# Autodesk Inventor assembly: Intake Pivot Encoder Mount
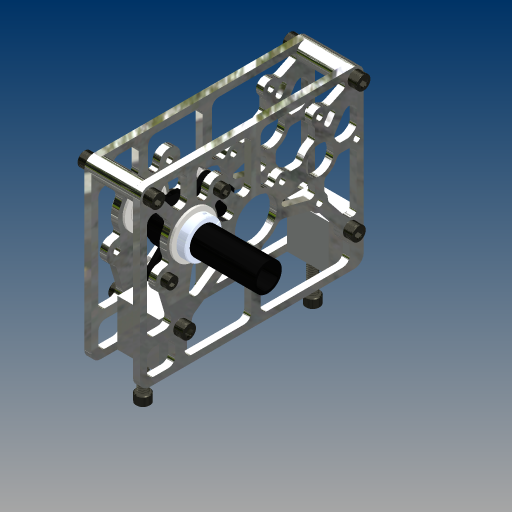
[picture p0: Inventor's stored thumbnail of the model, 512x512]
Saved by Autodesk Inventor 2024.3 (Build 283343000, 343)
## iProperties
Created: 2024-08-03
Part Number: Intake Pivot Encoder Mount
Document SubType Name: Assembly
Designer: Kenji
Author: Kenji
## Documents named in this file (15)
- C:\Users\Kenji\Documents\GitHub\1622-2024-Summer-CAD-A-Thon\Intake\Intake Pivot Encoder Mount.iam
- C:\Users\Kenji\Documents\GitHub\1622-2024-Summer-CAD-A-Thon\Intake\Intake Pivot Gearbox Plate.ipt
- C:\Users\Kenji\Documents\GitHub\1622-2024-Summer-CAD-A-Thon\Intake\Intake Pivot Spacer 3.ipt
- C:\Users\Kenji\Documents\GitHub\1622-2024-Summer-CAD-A-Thon\Intake\Intake Pivot Billet.ipt
- C:\Users\Kenji\Documents\GitHub\1622-2024-Summer-CAD-A-Thon\COTS Library\Fasteners\Bolts\Socket-Head\0.25-20\COTS_91251A539_Black-Oxide Alloy Steel Socket Head Screw (1).ipt
- C:\Users\Kenji\Documents\GitHub\1622-2024-Summer-CAD-A-Thon\COTS Library\Motion\Bearings\COTS_WCP-0783_1.125ODHexBearing.ipt
- C:\Users\Kenji\Documents\GitHub\1622-2024-Summer-CAD-A-Thon\COTS Library\Fasteners\Bolts\Button-Head\0.25-20\COTS_0.25-20_ButtonHead_0.5inlong_StainlessSteel_92949A537.ipt
- C:\Users\Kenji\Documents\GitHub\1622-2024-Summer-CAD-A-Thon\COTS Library\Fasteners\Washers\COTS_90107A029_316 Stainless Steel Washer.ipt
- C:\Users\Kenji\Documents\GitHub\1622-2024-Summer-CAD-A-Thon\Intake\REV-11-1271(ThroughBoreEncoder).iam
- C:\Users\Kenji\Documents\GitHub\1622-2024-Summer-CAD-A-Thon\COTS Library\Fasteners\Nuts\COTS_90631A411_10-32_Nylock_Nut.ipt
- C:\Users\Kenji\Documents\GitHub\1622-2024-Summer-CAD-A-Thon\COTS Library\Fasteners\Washers\COTS_91860A047_Size10Washer.ipt
- C:\Users\Kenji\Documents\GitHub\1622-2024-Summer-CAD-A-Thon\COTS Library\Fasteners\Bolts\Socket-Head\10-32\COTS_91251A345_Black-Oxide Alloy Steel Socket Head Screw.ipt
- C:\Users\Kenji\Documents\GitHub\1622-2024-Summer-CAD-A-Thon\COTS Library\Fasteners\Shaft Collars\COTS_WCP-0799_0.5inchHexShaftCollar.ipt
- C:\Users\Kenji\Documents\GitHub\1622-2024-Summer-CAD-A-Thon\Intake\Intake Pivot Spacer 4.ipt
- C:\Users\Kenji\Documents\GitHub\1622-2024-Summer-CAD-A-Thon\COTS Library\Fasteners\Bolts\Socket-Head\0.25-20\COTS_90044A123_Black-Oxide Alloy Steel Socket Head Screw.ipt
## Components (29 placed, 14 different names)
1. Intake Pivot Gearbox Plate:1 — Mate:1, Mate:2, Mate:3, Mate:4, Mate:6, Mate:9, Flush:1, Flush:2, Mate:13, Mate:14, Mate:18, Mate:19, Mate:21, Mate:22, Mate:26, Mate:27, Mate:28, Mate:29
2. Intake Pivot Gearbox Plate:2 — Mate:1, Mate:2, Mate:5, Mate:7, Mate:8, Mate:10, Mate:11, Mate:12, Mate:15, Mate:16, Mate:17, Mate:20, Mate:23, Mate:24, Mate:25, Mate:34, Mate:35, Mate:36, Mate:45, Mate:46, Mate:51, Mate:52, Mate:53, Mate:54, Mate:55, Mate:56
3. Intake Pivot Spacer 3:1 — Mate:3, Mate:4, Mate:5
4. Intake Pivot Spacer 3:2 — Mate:6, Mate:7
5. Intake Pivot Billet:1 — Mate:10, Flush:2, Mate:11, Mate:61, Mate:64
6. Intake Pivot Billet:2 — Mate:8, Mate:9, Flush:1, Mate:62, Mate:63
7. COTS_91251A539_Black-Oxide Alloy Steel Socket Head Screw (1):1 — Mate:13, Mate:18
8. COTS_91251A539_Black-Oxide Alloy Steel Socket Head Screw (1):2 — Mate:15, Mate:16
9. COTS_91251A539_Black-Oxide Alloy Steel Socket Head Screw (1):3 — Mate:12, Mate:17
10. COTS_91251A539_Black-Oxide Alloy Steel Socket Head Screw (1):4 — Mate:14, Mate:19
11. COTS_91251A539_Black-Oxide Alloy Steel Socket Head Screw (1):5 — Mate:22, Mate:27
12. COTS_91251A539_Black-Oxide Alloy Steel Socket Head Screw (1):6 — Mate:23, Mate:24
13. COTS_91251A539_Black-Oxide Alloy Steel Socket Head Screw (1):7 — Mate:21, Mate:26
14. COTS_91251A539_Black-Oxide Alloy Steel Socket Head Screw (1):8 — Mate:20, Mate:25
15. COTS_WCP-0783_1.125ODHexBearing:1 — Mate:28, Mate:29, Mate:30, Mate:31
16. COTS_0.25-20_ButtonHead_0.5inlong_StainlessSteel_92949A537:1 — Mate:32, Mate:33
17. COTS_90107A029_316 Stainless Steel Washer:1 — Mate:30, Mate:31, Mate:32, Mate:33
18. REV-11-1271(ThroughBoreEncoder):1 [sub-assembly] — Mate:34, Mate:35, Mate:36, Mate:42, Mate:44
19. COTS_90631A411_10-32_Nylock_Nut:1 — Mate:49, Mate:50
20. COTS_90631A411_10-32_Nylock_Nut:2 — Mate:47, Mate:48
21. COTS_91860A047_Size10Washer:1 — Mate:42, Mate:45, Mate:49, Mate:50
22. COTS_91860A047_Size10Washer:2 — Mate:44, Mate:46, Mate:47, Mate:48
23. COTS_91251A345_Black-Oxide Alloy Steel Socket Head Screw:1 — Mate:52, Mate:54
24. COTS_91251A345_Black-Oxide Alloy Steel Socket Head Screw:2 — Mate:51, Mate:53
25. COTS_WCP-0783_1.125ODHexBearing:2 — Mate:55, Mate:56, Mate:57, Mate:58
26. COTS_WCP-0799_0.5inchHexShaftCollar:1 — Mate:57, Mate:58, Mate:59, Mate:60
27. Intake Pivot Spacer 4:1 — Mate:59, Mate:60
28. COTS_90044A123_Black-Oxide Alloy Steel Socket Head Screw:1 — Mate:61, Mate:64
29. COTS_90044A123_Black-Oxide Alloy Steel Socket Head Screw:2 — Mate:62, Mate:63
## Relationships (60: Mate 58, Flush 2)
- Mate:1: Intake Pivot Gearbox Plate:1 ↔ Intake Pivot Gearbox Plate:2
- Mate:2: Intake Pivot Gearbox Plate:1 ↔ Intake Pivot Gearbox Plate:2
- Mate:3: Intake Pivot Gearbox Plate:1 ↔ Intake Pivot Spacer 3:1
- Mate:4: Intake Pivot Gearbox Plate:1 ↔ Intake Pivot Spacer 3:1
- Mate:5: Intake Pivot Gearbox Plate:2 ↔ Intake Pivot Spacer 3:1
- Mate:6: Intake Pivot Gearbox Plate:1 ↔ Intake Pivot Spacer 3:2
- Mate:7: Intake Pivot Gearbox Plate:2 ↔ Intake Pivot Spacer 3:2
- Mate:8: Intake Pivot Gearbox Plate:2 ↔ Intake Pivot Billet:2
- Mate:9: Intake Pivot Gearbox Plate:1 ↔ Intake Pivot Billet:2
- Flush:1: Intake Pivot Gearbox Plate:1 ↔ Intake Pivot Billet:2
- Mate:10: Intake Pivot Gearbox Plate:2 ↔ Intake Pivot Billet:1
- Flush:2: Intake Pivot Gearbox Plate:1 ↔ Intake Pivot Billet:1
- Mate:11: Intake Pivot Gearbox Plate:2 ↔ Intake Pivot Billet:1
- Mate:12: Intake Pivot Gearbox Plate:2 ↔ COTS_91251A539_Black-Oxide Alloy Steel Socket Head Screw (1):3
- Mate:13: Intake Pivot Gearbox Plate:1 ↔ COTS_91251A539_Black-Oxide Alloy Steel Socket Head Screw (1):1
- Mate:14: Intake Pivot Gearbox Plate:1 ↔ COTS_91251A539_Black-Oxide Alloy Steel Socket Head Screw (1):4
- Mate:15: Intake Pivot Gearbox Plate:2 ↔ COTS_91251A539_Black-Oxide Alloy Steel Socket Head Screw (1):2
- Mate:16: Intake Pivot Gearbox Plate:2 ↔ COTS_91251A539_Black-Oxide Alloy Steel Socket Head Screw (1):2
- Mate:17: Intake Pivot Gearbox Plate:2 ↔ COTS_91251A539_Black-Oxide Alloy Steel Socket Head Screw (1):3
- Mate:18: Intake Pivot Gearbox Plate:1 ↔ COTS_91251A539_Black-Oxide Alloy Steel Socket Head Screw (1):1
- Mate:19: Intake Pivot Gearbox Plate:1 ↔ COTS_91251A539_Black-Oxide Alloy Steel Socket Head Screw (1):4
- Mate:20: Intake Pivot Gearbox Plate:2 ↔ COTS_91251A539_Black-Oxide Alloy Steel Socket Head Screw (1):8
- Mate:21: Intake Pivot Gearbox Plate:1 ↔ COTS_91251A539_Black-Oxide Alloy Steel Socket Head Screw (1):7
- Mate:22: Intake Pivot Gearbox Plate:1 ↔ COTS_91251A539_Black-Oxide Alloy Steel Socket Head Screw (1):5
- Mate:23: Intake Pivot Gearbox Plate:2 ↔ COTS_91251A539_Black-Oxide Alloy Steel Socket Head Screw (1):6
- Mate:24: Intake Pivot Gearbox Plate:2 ↔ COTS_91251A539_Black-Oxide Alloy Steel Socket Head Screw (1):6
- Mate:25: Intake Pivot Gearbox Plate:2 ↔ COTS_91251A539_Black-Oxide Alloy Steel Socket Head Screw (1):8
- Mate:26: Intake Pivot Gearbox Plate:1 ↔ COTS_91251A539_Black-Oxide Alloy Steel Socket Head Screw (1):7
- Mate:27: Intake Pivot Gearbox Plate:1 ↔ COTS_91251A539_Black-Oxide Alloy Steel Socket Head Screw (1):5
- Mate:28: Intake Pivot Gearbox Plate:1 ↔ COTS_WCP-0783_1.125ODHexBearing:1
- Mate:29: Intake Pivot Gearbox Plate:1 ↔ COTS_WCP-0783_1.125ODHexBearing:1
- Mate:30: COTS_WCP-0783_1.125ODHexBearing:1 ↔ COTS_90107A029_316 Stainless Steel Washer:1
- Mate:31: COTS_WCP-0783_1.125ODHexBearing:1 ↔ COTS_90107A029_316 Stainless Steel Washer:1
- Mate:32: COTS_0.25-20_ButtonHead_0.5inlong_StainlessSteel_92949A537:1 ↔ COTS_90107A029_316 Stainless Steel Washer:1
- Mate:33: COTS_0.25-20_ButtonHead_0.5inlong_StainlessSteel_92949A537:1 ↔ COTS_90107A029_316 Stainless Steel Washer:1
- Mate:34: Intake Pivot Gearbox Plate:2 ↔ REV-11-1271(ThroughBoreEncoder):1
- Mate:35: Intake Pivot Gearbox Plate:2 ↔ REV-11-1271(ThroughBoreEncoder):1
- Mate:36: Intake Pivot Gearbox Plate:2 ↔ REV-11-1271(ThroughBoreEncoder):1
- Mate:42: REV-11-1271(ThroughBoreEncoder):1 ↔ COTS_91860A047_Size10Washer:1
- Mate:44: REV-11-1271(ThroughBoreEncoder):1 ↔ COTS_91860A047_Size10Washer:2
- Mate:45: Intake Pivot Gearbox Plate:2 ↔ COTS_91860A047_Size10Washer:1
- Mate:46: Intake Pivot Gearbox Plate:2 ↔ COTS_91860A047_Size10Washer:2
- Mate:47: COTS_90631A411_10-32_Nylock_Nut:2 ↔ COTS_91860A047_Size10Washer:2
- Mate:48: COTS_90631A411_10-32_Nylock_Nut:2 ↔ COTS_91860A047_Size10Washer:2
- Mate:49: COTS_90631A411_10-32_Nylock_Nut:1 ↔ COTS_91860A047_Size10Washer:1
- Mate:50: COTS_90631A411_10-32_Nylock_Nut:1 ↔ COTS_91860A047_Size10Washer:1
- Mate:51: Intake Pivot Gearbox Plate:2 ↔ COTS_91251A345_Black-Oxide Alloy Steel Socket Head Screw:2
- Mate:52: Intake Pivot Gearbox Plate:2 ↔ COTS_91251A345_Black-Oxide Alloy Steel Socket Head Screw:1
- Mate:53: Intake Pivot Gearbox Plate:2 ↔ COTS_91251A345_Black-Oxide Alloy Steel Socket Head Screw:2
- Mate:54: Intake Pivot Gearbox Plate:2 ↔ COTS_91251A345_Black-Oxide Alloy Steel Socket Head Screw:1
- Mate:55: Intake Pivot Gearbox Plate:2 ↔ COTS_WCP-0783_1.125ODHexBearing:2
- Mate:56: Intake Pivot Gearbox Plate:2 ↔ COTS_WCP-0783_1.125ODHexBearing:2
- Mate:57: COTS_WCP-0783_1.125ODHexBearing:2 ↔ COTS_WCP-0799_0.5inchHexShaftCollar:1
- Mate:58: COTS_WCP-0783_1.125ODHexBearing:2 ↔ COTS_WCP-0799_0.5inchHexShaftCollar:1
- Mate:59: COTS_WCP-0799_0.5inchHexShaftCollar:1 ↔ Intake Pivot Spacer 4:1
- Mate:60: COTS_WCP-0799_0.5inchHexShaftCollar:1 ↔ Intake Pivot Spacer 4:1
- Mate:61: Intake Pivot Billet:1 ↔ COTS_90044A123_Black-Oxide Alloy Steel Socket Head Screw:1
- Mate:62: Intake Pivot Billet:2 ↔ COTS_90044A123_Black-Oxide Alloy Steel Socket Head Screw:2
- Mate:63 (25.4 mm): Intake Pivot Billet:2 ↔ COTS_90044A123_Black-Oxide Alloy Steel Socket Head Screw:2
- Mate:64 (25.4 mm): Intake Pivot Billet:1 ↔ COTS_90044A123_Black-Oxide Alloy Steel Socket Head Screw:1
